# Autodesk Inventor assembly: strut
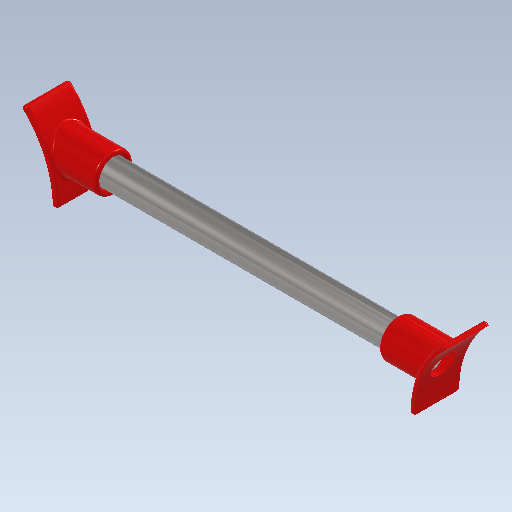
[picture p0: Inventor's stored thumbnail of the model, 512x512]
Saved by Autodesk Inventor 2020.2 (Build 242310000, 310)
## iProperties
Created: 2020-03-22
Part Number: strut
Document SubType Name: Assembly
Designer: agmle
Mass: 451.216 g
Surface Area: 1082.2 cm^2
Volume: 158.09 cm^3
Density: 2.85417 g/cm^3
Author: agmle
## Documents named in this file (3)
- D:\projects\CreekFleet_AutoBuoy\Mechanical CAD\hull\strut.iam
- D:\projects\CreekFleet_AutoBuoy\Mechanical CAD\hull\strut.ipt
- D:\projects\CreekFleet_AutoBuoy\Mechanical CAD\hull\strut_flange.ipt
## Components (3 placed, 2 different names)
1. strut:1 — Insert:1, Insert:2
2. strut_flange:1 — Insert:1, Flush:1, Mate:1, Mate:2
3. strut_flange:2 — Insert:2, Flush:1
## Relationships (5: Insert 2, Mate 2, Flush 1)
- Insert:1: strut:1 ↔ strut_flange:1
- Insert:2: strut:1 ↔ strut_flange:2
- Flush:1: strut_flange:1 ↔ strut_flange:2
- Mate:1: strut_flange:1
- Mate:2: strut_flange:1
